# Autodesk Inventor assembly: Assembly_HITscope
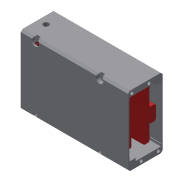
[picture p0: Inventor's stored thumbnail of the model, 180x180]
Saved by Autodesk Inventor 2019 (Build 230136000, 136)
## iProperties
Created: 2021-09-09
Part Number: Assembly_HITscope
Material: Generisch
Document SubType Name: Assembly
Designer: Muriel
Author: Muriel
## Documents named in this file (4)
- C:\Users\Muriel\Documents\Inventor\HITscope\Assembly_HITscope.iam
- C:\Users\Muriel\Documents\Inventor\HITscope\HITscope_v0.iam
- C:\Users\Muriel\Documents\Inventor\HITscope\02_Camera_Module_Lid_v0.ipt
- C:\Users\Muriel\Documents\Inventor\Content Center Files\R2019\de-DE\DIN 912\DIN 912 - M3 x 0,5 x 8 x 6,75.ipt
## Components (7 placed, 3 different names)
1. 02_Camera_Module_Lid_v0:1 — Einfügen:1, Einfügen:2, Einfügen:3, Einfügen:4
2. DIN 912 - ersetzt durch DIN EN ISO 4762 M3 x 8:1 — Einfügen:1
3. DIN 912 - ersetzt durch DIN EN ISO 4762 M3 x 8:2 — Einfügen:2
4. DIN 912 - ersetzt durch DIN EN ISO 4762 M3 x 8:3 — Einfügen:3
5. DIN 912 - ersetzt durch DIN EN ISO 4762 M3 x 8:4 — Einfügen:4
6. HITscope_v0:4 [sub-assembly] — Passend:1, Fluchtend:1, Fluchtend:2
7. HITscope_v0:5 [sub-assembly] — Passend:1, Fluchtend:1, Fluchtend:2
## Relationships (7: Insert 4, Flush 2, Mate 1)
- Einfügen:1 [Insert]: 02_Camera_Module_Lid_v0:1 ↔ DIN 912 - ersetzt durch DIN EN ISO 4762 M3 x 8:1
- Einfügen:2 [Insert]: 02_Camera_Module_Lid_v0:1 ↔ DIN 912 - ersetzt durch DIN EN ISO 4762 M3 x 8:2
- Einfügen:3 [Insert]: 02_Camera_Module_Lid_v0:1 ↔ DIN 912 - ersetzt durch DIN EN ISO 4762 M3 x 8:3
- Einfügen:4 [Insert]: 02_Camera_Module_Lid_v0:1 ↔ DIN 912 - ersetzt durch DIN EN ISO 4762 M3 x 8:4
- Passend:1 [Mate]: HITscope_v0:4 ↔ HITscope_v0:5
- Fluchtend:1 [Flush]: HITscope_v0:4 ↔ HITscope_v0:5
- Fluchtend:2 [Flush]: HITscope_v0:4 ↔ HITscope_v0:5
